# Autodesk Inventor assembly: hardstop
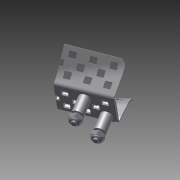
[picture p0: Inventor's stored thumbnail of the model, 180x180]
Saved by Autodesk Inventor 2014 SP1 (Build 180222100, 222)
## iProperties
Created: 2014-04-06
Part Number: hardstop
Document SubType Name: Assembly
Designer: Ryan
Author: Ryan
## Documents named in this file (6)
- C:\Users\Ryan\Desktop\sw\toss up 5th A bot\drive\hardstop.iam
- C:\Users\Ryan\Desktop\sw\lib\Aperture VEX CAD Library\Metal\L Bar\2 x 3 bent for 169A rev5 hardstop.ipt
- C:\Users\Ryan\Desktop\sw\lib\Aperture VEX CAD Library\Metal\L Bar\2 x 3 bent for 169A rev5 hardstop_MIR.ipt
- C:\Users\Ryan\Desktop\sw\lib\Aperture VEX CAD Library\Spacers\thin\SPACER-0320-0500.ipt
- C:\Users\Ryan\Desktop\sw\lib\Aperture VEX CAD Library\Hardware\8-32\8-32_.875.ipt
- C:\Users\Ryan\Desktop\sw\lib\Aperture VEX CAD Library\Hardware\8-32\8-32 nylock.ipt
## Components (8 placed, 5 different names)
1. 2 x 3 bent for 169A rev5 hardstop:1 — Mate:1, Flush:1, Flush:2, Mate:2, Mate:5, Mate:7, Mate:9, Mate:11
2. 2 x 3 bent for 169A rev5 hardstop_MIR:1 — Mate:1, Flush:1, Flush:2, Mate:3, Mate:4, Mate:6
3. SPACER-0320-0500:1 — Mate:2, Mate:3, Mate:4, Mate:10, Mate:15
4. SPACER-0320-0500:2 — Mate:5, Mate:6, Mate:7, Mate:8, Mate:13
5. 8-32_.875:1 — Mate:8, Mate:9, Mate:12
6. 8-32_.875:2 — Mate:10, Mate:11, Mate:14
7. 8-32 nylock:1 — Mate:12, Mate:13
8. 8-32 nylock:2 — Mate:14, Mate:15
## Relationships (17: Mate 15, Flush 2)
- Mate:1: 2 x 3 bent for 169A rev5 hardstop:1 ↔ 2 x 3 bent for 169A rev5 hardstop_MIR:1
- Flush:1: 2 x 3 bent for 169A rev5 hardstop:1 ↔ 2 x 3 bent for 169A rev5 hardstop_MIR:1
- Flush:2: 2 x 3 bent for 169A rev5 hardstop:1 ↔ 2 x 3 bent for 169A rev5 hardstop_MIR:1
- Mate:2 (2.3114 mm): 2 x 3 bent for 169A rev5 hardstop:1 ↔ SPACER-0320-0500:1
- Mate:3: 2 x 3 bent for 169A rev5 hardstop_MIR:1 ↔ SPACER-0320-0500:1
- Mate:4 (2.3114 mm): 2 x 3 bent for 169A rev5 hardstop_MIR:1 ↔ SPACER-0320-0500:1
- Mate:5 (2.3114 mm): 2 x 3 bent for 169A rev5 hardstop:1 ↔ SPACER-0320-0500:2
- Mate:6: 2 x 3 bent for 169A rev5 hardstop_MIR:1 ↔ SPACER-0320-0500:2
- Mate:7 (2.3114 mm): 2 x 3 bent for 169A rev5 hardstop:1 ↔ SPACER-0320-0500:2
- Mate:8: SPACER-0320-0500:2 ↔ 8-32_.875:1
- Mate:9: 2 x 3 bent for 169A rev5 hardstop:1 ↔ 8-32_.875:1
- Mate:10: SPACER-0320-0500:1 ↔ 8-32_.875:2
- Mate:11: 2 x 3 bent for 169A rev5 hardstop:1 ↔ 8-32_.875:2
- Mate:12: 8-32_.875:1 ↔ 8-32 nylock:1
- Mate:13 (1.1684 mm): SPACER-0320-0500:2 ↔ 8-32 nylock:1
- Mate:14: 8-32_.875:2 ↔ 8-32 nylock:2
- Mate:15 (1.1684 mm): SPACER-0320-0500:1 ↔ 8-32 nylock:2
## Named parameters: q = 2.3114 mm
